# Autodesk Inventor assembly: Main Carriage
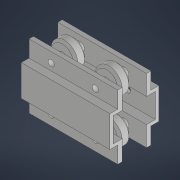
[picture p0: Inventor's stored thumbnail of the model, 180x180]
Saved by Autodesk Inventor 2022 (Build 260153000, 153)
## iProperties
Created: 2023-06-23
Part Number: Main Carriage
Document SubType Name: Assembly
Designer: Ryan Mitcham
Author: Ryan Mitcham
## Documents named in this file (4)
- C:\Users\Gaming\OneDrive\Documents\Inventor\XYZ-Gantry\Main Carriage\Main Carriage.iam
- C:\Users\Gaming\OneDrive\Documents\Inventor\XYZ-Gantry\Main Carriage\Wheel Base.ipt
- C:\Users\Gaming\OneDrive\Documents\Inventor\XYZ-Gantry\Standard Parts\20x20 Extrusion Compatible Wheel - Dual Spacers.ipt
- C:\Users\Gaming\OneDrive\Documents\Inventor\XYZ-Gantry\Main Carriage\Wheel Base - No Belt Clamp.ipt
## Components (6 placed, 3 different names)
1. Wheel Base:1 — Mate:1, Mate:2, Mate:3, Mate:4, Mate:5, Mate:6, Mate:7, Mate:8, Mate:9, Mate:10, Mate:11
2. 20x20 Extrusion Compatible Wheel - Dual Spacers:1 — Mate:1, Mate:5, Mate:12, Mate:14
3. 20x20 Extrusion Compatible Wheel - Dual Spacers:2 — Mate:2, Mate:6
4. 20x20 Extrusion Compatible Wheel - Dual Spacers:3 — Mate:4, Mate:8
5. 20x20 Extrusion Compatible Wheel - Dual Spacers:4 — Mate:3, Mate:7, Mate:13
6. Wheel Base - No Belt Clamp:1 — Mate:12, Mate:13, Mate:14
## Relationships (14: Mate 14)
- Mate:1: Wheel Base:1 ↔ 20x20 Extrusion Compatible Wheel - Dual Spacers:1
- Mate:2: Wheel Base:1 ↔ 20x20 Extrusion Compatible Wheel - Dual Spacers:2
- Mate:3: Wheel Base:1 ↔ 20x20 Extrusion Compatible Wheel - Dual Spacers:4
- Mate:4: Wheel Base:1 ↔ 20x20 Extrusion Compatible Wheel - Dual Spacers:3
- Mate:5: Wheel Base:1 ↔ 20x20 Extrusion Compatible Wheel - Dual Spacers:1
- Mate:6: Wheel Base:1 ↔ 20x20 Extrusion Compatible Wheel - Dual Spacers:2
- Mate:7: Wheel Base:1 ↔ 20x20 Extrusion Compatible Wheel - Dual Spacers:4
- Mate:8: Wheel Base:1 ↔ 20x20 Extrusion Compatible Wheel - Dual Spacers:3
- Mate:9: Wheel Base:1
- Mate:10: Wheel Base:1
- Mate:11: Wheel Base:1
- Mate:12: 20x20 Extrusion Compatible Wheel - Dual Spacers:1 ↔ Wheel Base - No Belt Clamp:1
- Mate:13: 20x20 Extrusion Compatible Wheel - Dual Spacers:4 ↔ Wheel Base - No Belt Clamp:1
- Mate:14: 20x20 Extrusion Compatible Wheel - Dual Spacers:1 ↔ Wheel Base - No Belt Clamp:1
